# Autodesk Inventor assembly: HbFinger_flex02
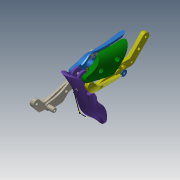
[picture p0: Inventor's stored thumbnail of the model, 180x180]
Saved by Autodesk Inventor 2015 SP1 (Build 190203100, 203)
## iProperties
Created: 2015-02-20
Part Number: HbFinger_flex02
Document SubType Name: Assembly
Designer: Yamaura
Author: Yamaura
## Documents named in this file (9)
- C:\Users\Yamaura\Documents\GitHub\HACKberry\HACKberry-hardware\3D\Inventor\Parts\HbFinger_flex02.iam
- C:\Users\Yamaura\Documents\GitHub\HACKberry\HACKberry-hardware\3D\Inventor\Parts\HbProximalPhalanxCover02.ipt
- C:\Users\Yamaura\Documents\GitHub\HACKberry\HACKberry-hardware\3D\Inventor\Parts\HbProximalPhalanx02.ipt
- C:\Users\Yamaura\Documents\GitHub\HACKberry\HACKberry-hardware\3D\Inventor\Parts\HbMiddle-DistalPhalanx02.ipt
- C:\Users\Yamaura\Documents\GitHub\HACKberry\HACKberry-hardware\3D\Inventor\Parts\HbCouplerLink02.ipt
- C:\Users\Yamaura\Documents\GitHub\HACKberry\HACKberry-hardware\3D\Inventor\Parts\HbFingerPosture_flex02.ipt
- C:\Users\Yamaura\Documents\GitHub\HACKberry\HACKberry-hardware\3D\Inventor\Parts\HbCouplerLinkCover03.ipt
- C:\Users\Yamaura\Documents\GitHub\HACKberry\HACKberry-hardware\3D\Inventor\Parts\ScrewM2L12.ipt
- C:\Users\Yamaura\Documents\GitHub\HACKberry\HACKberry-hardware\3D\Inventor\Parts\MetalCollarPh3L5.ipt
## Components (8 placed, 8 different names)
1. HbFingerPosture01:1 — フラッシュ:14, フラッシュ:15, フラッシュ:16, メイト:4, メイト:8, メイト:13, メイト:14, メイト:15, メイト:18, メイト:19, メイト:27, メイト:28
2. HbMiddle-DistalPhalanx02:1 — フラッシュ:1, メイト:4, メイト:18
3. HbProximalPhalanx02:1 — フラッシュ:12, メイト:23, メイト:25, メイト:27, メイト:28
4. HbProximalPhalanxCover02:1 — フラッシュ:17, メイト:13, メイト:14, メイト:22
5. HbCouplerLink02:1 — フラッシュ:13, メイト:8, メイト:15, メイト:20, メイト:21
6. HbCouplerLinkCover03:1 — メイト:19, メイト:20, メイト:21
7. ScrewM2L12:1 — メイト:22, メイト:23, メイト:24
8. MetalCollarPh3L5:1 — メイト:24, メイト:25
## Relationships (22: Mate 15, Flush 7)
- フラッシュ:1 [Flush]: HbMiddle-DistalPhalanx02:1
- フラッシュ:12 [Flush]: HbProximalPhalanx02:1
- フラッシュ:13 [Flush]: HbCouplerLink02:1
- フラッシュ:14 [Flush]: HbFingerPosture01:1
- フラッシュ:15 [Flush]: HbFingerPosture01:1
- フラッシュ:16 [Flush]: HbFingerPosture01:1
- メイト:4 [Mate]: HbFingerPosture01:1 ↔ HbMiddle-DistalPhalanx02:1
- メイト:8 [Mate]: HbFingerPosture01:1 ↔ HbCouplerLink02:1
- フラッシュ:17 [Flush]: HbProximalPhalanxCover02:1
- メイト:13 [Mate]: HbFingerPosture01:1 ↔ HbProximalPhalanxCover02:1
- メイト:14 [Mate]: HbFingerPosture01:1 ↔ HbProximalPhalanxCover02:1
- メイト:15 [Mate]: HbFingerPosture01:1 ↔ HbCouplerLink02:1
- メイト:18 [Mate]: HbFingerPosture01:1 ↔ HbMiddle-DistalPhalanx02:1
- メイト:19 [Mate]: HbFingerPosture01:1 ↔ HbCouplerLinkCover03:1
- メイト:20 [Mate]: HbCouplerLink02:1 ↔ HbCouplerLinkCover03:1
- メイト:21 [Mate]: HbCouplerLink02:1 ↔ HbCouplerLinkCover03:1
- メイト:22 [Mate]: HbProximalPhalanxCover02:1 ↔ ScrewM2L12:1
- メイト:23 [Mate]: HbProximalPhalanx02:1 ↔ ScrewM2L12:1
- メイト:24 [Mate]: ScrewM2L12:1 ↔ MetalCollarPh3L5:1
- メイト:25 [Mate] (0.25 mm): HbProximalPhalanx02:1 ↔ MetalCollarPh3L5:1
- メイト:27 [Mate]: HbFingerPosture01:1 ↔ HbProximalPhalanx02:1
- メイト:28 [Mate]: HbFingerPosture01:1 ↔ HbProximalPhalanx02:1
